# Autodesk Inventor assembly: MGN-12H
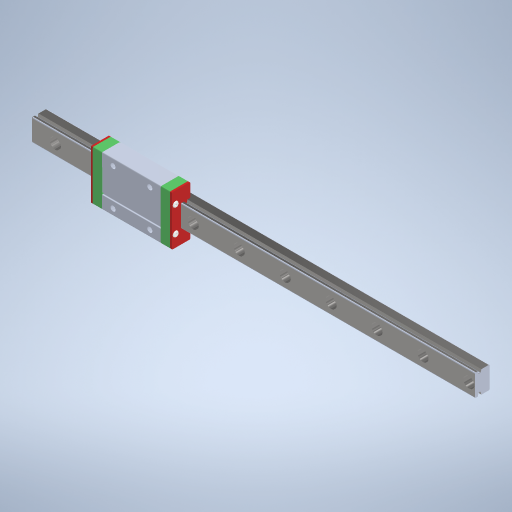
[picture p0: Inventor's stored thumbnail of the model, 512x512]
Saved by Autodesk Inventor 2023.1 (Build 271208000, 208)
## iProperties
Created: 2021-10-05
Part Number: MGN-12H
Document SubType Name: Assembly
Designer: nicol
Author: nicol
## Documents named in this file (6)
- Y:\Projects\T_Bot_Printer\MGN-12H\MGN-12H.iam
- Y:\Projects\Bibble0\Hardware\MGN-12H\Button M3x8.ipt
- Y:\Projects\Bibble0\Hardware\MGN-12H\Green End Cap.ipt
- Y:\Projects\Bibble0\Hardware\MGN-12H\Main Block.ipt
- Y:\Projects\Bibble0\Hardware\MGN-12H\Red End Cap.ipt
- Y:\Projects\Bibble0\Hardware\MGN-12H\Rail 400mm.ipt
## Components (10 placed, 5 different names)
1. Button M3x8:1 — Insert:12
2. Green End Cap:1 — Insert:1, Insert:2, Insert:3, Insert:4
3. Main Block:1 — Insert:1, Insert:2, Insert:5, Insert:6, Mate:1, Mate:2
4. Green End Cap:2 — Insert:5, Insert:6, Insert:7, Insert:8
5. Red End Cap:1 — Insert:3, Insert:4, Insert:11, Insert:12
6. Red End Cap:2 — Insert:7, Insert:8, Insert:9, Insert:10, Flush:1
7. Button M3x8:2 — Insert:9
8. Button M3x8:3 — Insert:10
9. Button M3x8:4 — Insert:11
10. Rail 400mm:1 — Mate:1, Mate:2, Flush:1
## Relationships (15: Insert 12, Mate 2, Flush 1)
- Insert:1: Green End Cap:1 ↔ Main Block:1
- Insert:2: Green End Cap:1 ↔ Main Block:1
- Insert:3: Green End Cap:1 ↔ Red End Cap:1
- Insert:4: Green End Cap:1 ↔ Red End Cap:1
- Insert:5: Main Block:1 ↔ Green End Cap:2
- Insert:6: Main Block:1 ↔ Green End Cap:2
- Insert:7: Green End Cap:2 ↔ Red End Cap:2
- Insert:8: Green End Cap:2 ↔ Red End Cap:2
- Insert:9: Red End Cap:2 ↔ Button M3x8:2
- Insert:10: Red End Cap:2 ↔ Button M3x8:3
- Insert:11: Red End Cap:1 ↔ Button M3x8:4
- Insert:12: Button M3x8:1 ↔ Red End Cap:1
- Mate:1: Main Block:1 ↔ Rail 400mm:1
- Mate:2: Main Block:1 ↔ Rail 400mm:1
- Flush:1: Red End Cap:2 ↔ Rail 400mm:1
